# Autodesk Inventor assembly: 4 mm
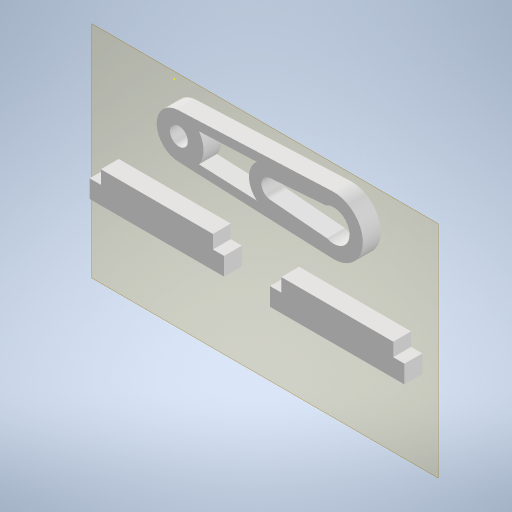
[picture p0: Inventor's stored thumbnail of the model, 512x512]
Saved by Autodesk Inventor 2023 (Build 270158000, 158)
## iProperties
Created: 2023-11-09
Part Number: 4 mm
Document SubType Name: Assembly
Designer: JULIAN
Author: JULIAN
## Documents named in this file (3)
- C:\Users\JULIAN\Desktop\Materias UN\Taller de Ingeniería Electrónica\Modelado cargo bot\DWG\4 mm.iam
- C:\Users\JULIAN\Desktop\Materias UN\Taller de Ingeniería Electrónica\Modelado cargo bot\Modelado\Aletas plato base.ipt
- C:\Users\JULIAN\Desktop\Materias UN\Taller de Ingeniería Electrónica\Modelado cargo bot\Modelado\Brazo conductor vertical 2.ipt
## Components (3 placed, 2 different names)
1. Aletas plato base:1 — Coincidencia:1
2. Brazo conductor vertical 2:1 — Coincidencia:3
3. Aletas plato base:2 — Coincidencia:2
## Relationships (3: Mate 3)
- Coincidencia:1 [Mate]: Aletas plato base:1
- Coincidencia:2 [Mate]: Aletas plato base:2
- Coincidencia:3 [Mate]: Brazo conductor vertical 2:1
